# Autodesk Inventor assembly: zlozenie
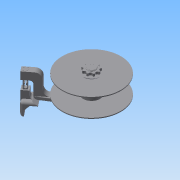
[picture p0: Inventor's stored thumbnail of the model, 180x180]
Saved by Autodesk Inventor 2017 (Build 210142000, 142)
## iProperties
Part Number: zlozenie
Material: Ogólny
Document SubType Name: Assembly
Designer: Kuba01
Author: Kuba01
## Documents named in this file (7)
- C:\Users\Kuba01\Desktop\3d print\uchyt na filament z waga\zlozenie.iam
- C:\Users\Kuba01\Desktop\3d print\uchyt na filament z waga\belka_tensometryczna.ipt
- C:\Users\Kuba01\Desktop\3d print\uchyt na filament z waga\mocowanie_do_ramy.ipt
- C:\Users\Kuba01\Desktop\3d print\uchyt na filament z waga\nakretka.ipt
- C:\Users\Kuba01\Desktop\3d print\uchyt na filament z waga\stożek.ipt
- C:\Users\Kuba01\Desktop\3d print\uchyt na filament z waga\uchwyt_filamentu.ipt
- C:\Users\Kuba01\Desktop\3d print\uchyt na filament z waga\szpula.ipt
## Components (7 placed, 6 different names)
1. belka_tensometryczna:1 — Zestawiający:1, Zestawiający:2, Zestawiający:3, Równoległy:1, Zestawiający:4, Zestawiający:5
2. mocowanie_do_ramy:1 — Zestawiający:1, Zestawiający:2, Zestawiający:3
3. nakretka:1 — Zestawiający:11, Zestawiający:12
4. stożek:1 — Zestawiający:6, Zestawiający:7
5. uchwyt_filamentu:1 — Równoległy:1, Zestawiający:4, Zestawiający:5, Zestawiający:6, Zestawiający:7, Zestawiający:8, Zestawiający:9, Zestawiający:10, Zestawiający:11
6. stożek:2 — Zestawiający:10, Równoległy:2, Zestawiający:12
7. szpula:1 — Zestawiający:8, Zestawiający:9, Równoległy:2
## Relationships (14: Mate 12, Flush 2)
- Zestawiający:1 [Mate] (1 mm): belka_tensometryczna:1 ↔ mocowanie_do_ramy:1
- Zestawiający:2 [Mate] (0.1 mm): belka_tensometryczna:1 ↔ mocowanie_do_ramy:1
- Zestawiający:3 [Mate] (0.1 mm): belka_tensometryczna:1 ↔ mocowanie_do_ramy:1
- Równoległy:1 [Flush]: belka_tensometryczna:1 ↔ uchwyt_filamentu:1
- Zestawiający:4 [Mate]: belka_tensometryczna:1 ↔ uchwyt_filamentu:1
- Zestawiający:5 [Mate] (0.1 mm): belka_tensometryczna:1 ↔ uchwyt_filamentu:1
- Zestawiający:6 [Mate]: stożek:1 ↔ uchwyt_filamentu:1
- Zestawiający:7 [Mate]: stożek:1 ↔ uchwyt_filamentu:1
- Zestawiający:8 [Mate]: uchwyt_filamentu:1 ↔ szpula:1
- Zestawiający:9 [Mate] (7 mm): uchwyt_filamentu:1 ↔ szpula:1
- Zestawiający:10 [Mate]: uchwyt_filamentu:1 ↔ stożek:2
- Równoległy:2 [Flush] (-7 mm): stożek:2 ↔ szpula:1
- Zestawiający:11 [Mate]: nakretka:1 ↔ uchwyt_filamentu:1
- Zestawiający:12 [Mate]: nakretka:1 ↔ stożek:2
